# Autodesk Inventor assembly: Microdrive_Compact_withCase
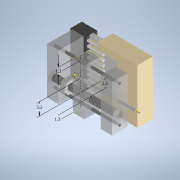
[picture p0: Inventor's stored thumbnail of the model, 180x180]
Saved by Autodesk Inventor 2020 (Build 240168000, 168)
## iProperties
Created: 2019-11-04
Part Number: Microdrive_Compact_withCase
Document SubType Name: Assembly
Designer: Knowblesse
Author: Knowblesse
## Documents named in this file (5)
- C:\VCF\Microdrive\Compact\Microdrive_Compact_withCase.iam
- C:\VCF\Microdrive\Compact\Microdrive_Compact.iam
- C:\VCF\Microdrive\Compact\PCB.ipt
- C:\VCF\Microdrive\Compact\PCB_Holder_Compact.ipt
- C:\VCF\Microdrive\Millmax.ipt
## Components (4 placed, 4 different names)
1. Microdrive_Compact:1 [sub-assembly] — 강체:3
2. PCB:1 — 강체:1, 강체:2
3. PCB_Holder_Compact:1 — 강체:1
4. Millmax:1 — 강체:2, 강체:3
## Relationships (3: WeldJoint 3)
- 강체:1 [WeldJoint]: PCB:1 ↔ PCB_Holder_Compact:1
- 강체:2 [WeldJoint]: PCB:1 ↔ Millmax:1
- 강체:3 [WeldJoint]: Microdrive_Compact:1 ↔ Millmax:1
